# Autodesk Inventor assembly: 左後脚ユニット5
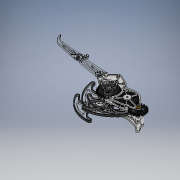
[picture p0: Inventor's stored thumbnail of the model, 180x180]
Saved by Autodesk Inventor 2020 (Build 240168000, 168)
## iProperties
Created: 2019-09-03
Part Number: 左後脚ユニット5
Document SubType Name: Assembly
Designer: 雪村
Mass: 251.015 g
Surface Area: 1556.42 cm^2
Volume: 120.818 cm^3
Density: 2.07763 g/cm^3
Author: 雪村
## Documents named in this file (29)
- C:\Users\white\Documents\SRDC\SRDC\Inventor_2017\2018年機体\2020年4年機体\左後脚ユニット5.iam
- C:\Users\white\Documents\SRDC\SRDC\Inventor_2017\2018年機体\2020年4年機体\脚クランク1.iam
- C:\Users\white\Documents\SRDC\SRDC\Inventor_2017\2018年機体\2020年4年機体\ヘッケン＋揺動節2.iam
- C:\Users\white\Documents\SRDC\SRDC\Inventor_2017\2018年機体\2020年4年機体\脚外フレーム5_MIR.ipt
- C:\Users\white\Documents\SRDC\SRDC\Inventor_2017\2018年機体\2020年4年機体\後脚ユニット締結パーツ5.ipt
- C:\Users\white\Documents\SRDC\SRDC\Inventor_2017\2018年機体\パーツ\スペーサーm3,40.ipt
- C:\Users\white\Documents\SRDC\SRDC\Inventor_2017\2018年機体\2020年4年機体\脚内フレーム5_MIR2.ipt
- C:\Users\white\Documents\SRDC\SRDC\Inventor_2017\2018年機体\2020年4年機体\脚最終段カム3.ipt
- C:\Users\white\Documents\SRDC\SRDC\Inventor_2017\2018年機体\パーツ\オイレスフランジ付き12142003.ipt
- C:\Users\white\Documents\SRDC\SRDC\Inventor_2017\2018年機体\パーツ\スペーサーm3,7.ipt
- C:\Users\white\Documents\SRDC\SRDC\Inventor_2017\2018年機体\2020年4年機体\歯車m2.z19.ipt
- C:\Users\white\Documents\SRDC\SRDC\Inventor_2017\2018年機体\パーツ\ベアリングフランジ付き0610.3t.ipt
- C:\Users\white\Documents\SRDC\SRDC\Inventor_2017\2018年機体\2020年4年機体\歯車m2.z25.ipt
- C:\Users\white\Documents\SRDC\SRDC\Inventor_2017\2018年機体\パーツ\オイレスフランジ付き06080512,1t ドライメット.ipt
- C:\Users\white\Documents\SRDC\SRDC\Inventor_2017\2018年機体\パーツ\スペーサーm3,6.ipt
- C:\Users\white\Documents\SRDC\SRDC\Inventor_2017\2018年機体\パーツ\ネジ鍋m3,12.ipt
- C:\Users\white\Documents\SRDC\SRDC\Inventor_2017\2018年機体\2020年4年機体\後脚ギアトレイン5.2.ipt
- C:\Users\white\Documents\SRDC\SRDC\Inventor_2017\2018年機体\2020年4年機体\歯車m2.z24.ipt
- C:\Users\white\Documents\SRDC\SRDC\Inventor_2017\2018年機体\2020年4年機体\後脚軸抑え1.ipt
- C:\Users\white\Documents\SRDC\SRDC\Inventor_2017\2018年機体\2020年4年機体\脚最終段カム4.ipt
- C:\Users\white\Documents\SRDC\SRDC\Inventor_2017\2018年機体\パーツ\スペーサーm3,4.ipt
- C:\Users\white\Documents\SRDC\SRDC\Inventor_2017\2018年機体\パーツ\ネジ皿m3,08.ipt
- C:\Users\white\Documents\SRDC\SRDC\Inventor_2017\2018年機体\パーツ\ネジ鍋m3,08.ipt
- C:\Users\white\Documents\SRDC\SRDC\Inventor_2017\2018年機体\パーツ\ネジ鍋m3,06.ipt
- C:\Users\white\Documents\SRDC\SRDC\Inventor_2017\2018年機体\パーツ\ネジ鍋m3,16.ipt
- C:\Users\white\Documents\SRDC\SRDC\Inventor_2017\2018年機体\2020年4年機体\後ウイング1.iam
- C:\Users\white\Documents\SRDC\SRDC\Inventor_2017\2018年機体\パーツ\スペーサーm3,20.ipt
- C:\Users\white\Documents\SRDC\SRDC\Inventor_2017\2018年機体\2020年4年機体\段ばね抑え2.ipt
- C:\Users\white\Documents\SRDC\SRDC\Inventor_2017\2018年機体\パーツ\スペーサーm3,5.ipt
## Components (75 placed, 28 different names)
1. 脚内フレーム5_MIR2:1 — 挿入:24, 挿入:25, 挿入:26, 挿入:27, 挿入:28, 挿入:39, 挿入:41, 挿入:43, 挿入:44, 挿入:45, 挿入:48, 挿入:62, 挿入:63, 挿入:64, 挿入:71, 挿入:72, 挿入:80, 挿入:85, 挿入:86, 挿入:87, 挿入:94
2. 脚クランク1:1 [sub-assembly] — 挿入:9, 挿入:10, 挿入:11, 挿入:12, 挿入:29, 挿入:30, 挿入:107
3. オイレスフランジ付き12142003:1 — 挿入:28
4. スペーサーm3,40:3 — 挿入:26
5. スペーサーm3,40:4 — 挿入:27, 挿入:70
6. スペーサーm3,40:2 — 挿入:25
7. スペーサーm3,40:1 — 挿入:24, 挿入:52, メイト:5
8. ヘッケン＋揺動節2:1 [sub-assembly] — 挿入:10
9. ヘッケン＋揺動節2:2 [sub-assembly] — 挿入:9
10. ヘッケン＋揺動節2:3 [sub-assembly] — 挿入:11
11. ヘッケン＋揺動節2:4 [sub-assembly] — 挿入:12
12. 脚外フレーム5_MIR:1 — 挿入:52, 挿入:70, 挿入:81, 挿入:82, 挿入:83, 挿入:84, 挿入:88, 挿入:106, 挿入:108
13. 後脚ユニット締結パーツ5:1 — メイト:5, 挿入:68, 挿入:69, 挿入:98, 挿入:99, 挿入:104, 挿入:105, 挿入:106
14. 脚最終段カム3:1 — 挿入:29, 挿入:30, 挿入:50, 挿入:51
15. スペーサーm3,7:1 — 挿入:48
16. スペーサーm3,7:2 — 挿入:39, 挿入:46
17. スペーサーm3,7:3 — 挿入:44
18. スペーサーm3,7:4 — 挿入:43
19. スペーサーm3,7:5 — 挿入:41, 挿入:47
20. 歯車m2.z19:1
21. ベアリングフランジ付き0610.3t:1
22. ベアリングフランジ付き0610.3t:2 — 挿入:72
23. 歯車m2.z25:1
24. ベアリングフランジ付き0610.3t:3 — 挿入:71
25. ベアリングフランジ付き0610.3t:4
26. オイレスフランジ付き06080512,1t ドライメット:1 — 挿入:45
27. オイレスフランジ付き06080512,1t ドライメット:2
28. スペーサーm3,6:1
29. スペーサーm3,6:2 — 挿入:49
30. ネジ鍋m3,12:1
31. ネジ鍋m3,12:2
32. 後脚ギアトレイン5.2:1 — 挿入:46, 挿入:47, 挿入:49, 挿入:73, 挿入:74, 挿入:75, 挿入:76
33. 歯車m2.z24:1 — 挿入:50, 挿入:51, 挿入:60, 挿入:61
34. 後脚軸抑え1:1 — 挿入:65, 挿入:66, 挿入:77, 挿入:78, 挿入:79
35. 脚最終段カム4:1 — 挿入:60, 挿入:61, 挿入:67, 挿入:89, 挿入:90, 挿入:91, 挿入:92
36. スペーサーm3,6:3 — 挿入:63, 挿入:66
37. スペーサーm3,6:4 — 挿入:62
38. スペーサーm3,6:5 — 挿入:64, 挿入:65
39. オイレスフランジ付き12142003:2 — 挿入:67
40. ベアリングフランジ付き0610.3t:5 — 挿入:68
41. スペーサーm3,4:1 — 挿入:69, 挿入:103
42. ネジ鍋m3,12:3 — 挿入:73
43. ネジ鍋m3,12:4 — 挿入:76
44. ネジ鍋m3,12:5 — 挿入:75
45. ネジ鍋m3,12:6 — 挿入:74
46. ネジ鍋m3,12:7 — 挿入:77
47. ネジ鍋m3,12:8 — 挿入:78
48. ネジ鍋m3,12:9 — 挿入:79
49. ネジ皿m3,08:1 — 挿入:80
50. ネジ鍋m3,08:1 — 挿入:86
51. ネジ鍋m3,08:2 — 挿入:87
52. ネジ鍋m3,08:3 — 挿入:85, 挿入:93
53. ネジ鍋m3,08:4 — 挿入:83
54. ネジ鍋m3,08:5 — 挿入:84
55. ネジ鍋m3,08:6 — 挿入:82
56. ネジ鍋m3,08:7 — 挿入:81
57. ネジ鍋m3,06:1 — 挿入:88
58. ネジ鍋m3,16:1 — 挿入:89
59. ネジ鍋m3,16:2 — 挿入:92
60. ネジ鍋m3,16:3 — 挿入:91
61. ネジ鍋m3,16:4 — 挿入:90
62. 後ウイング1:1 [sub-assembly] — 挿入:93
63. スペーサーm3,6:6 — 挿入:94
64. スペーサーm3,20:1 — 挿入:99
65. スペーサーm3,20:2
66. スペーサーm3,20:3 — 挿入:98
67. 段ばね抑え2:1 — 挿入:100, 挿入:101, 挿入:102
68. ネジ鍋m3,08:8 — 挿入:101
69. ネジ鍋m3,08:9 — 挿入:100
70. ネジ鍋m3,08:10 — 挿入:102
71. ネジ鍋m3,12:10 — 挿入:103
72. ネジ皿m3,08:2 — 挿入:104
73. ネジ皿m3,08:3 — 挿入:105
74. ベアリングフランジ付き0610.3t:6 — 挿入:108
75. スペーサーm3,5:1 — 挿入:107
## Relationships (86: Insert 81, Mate 5)
- [Insert]: 脚クランク1:1 ↔ オイレスフランジ付き12142003:1
- 挿入:9 [Insert] (0.5 mm): 脚クランク1:1 ↔ ヘッケン＋揺動節2:2
- 挿入:10 [Insert] (0.5 mm): 脚クランク1:1 ↔ ヘッケン＋揺動節2:1
- 挿入:11 [Insert] (0.5 mm): 脚クランク1:1 ↔ ヘッケン＋揺動節2:3
- 挿入:12 [Insert] (0.5 mm): 脚クランク1:1 ↔ ヘッケン＋揺動節2:4
- [Mate]: スペーサーm3,40:1 ↔ ヘッケン＋揺動節2:2
- [Mate]: スペーサーm3,40:1 ↔ ヘッケン＋揺動節2:1
- [Mate]: スペーサーm3,40:1 ↔ ヘッケン＋揺動節2:4
- [Mate]: スペーサーm3,40:1 ↔ ヘッケン＋揺動節2:3
- 挿入:24 [Insert]: 脚内フレーム5_MIR2:1 ↔ スペーサーm3,40:1
- 挿入:25 [Insert]: 脚内フレーム5_MIR2:1 ↔ スペーサーm3,40:2
- 挿入:26 [Insert]: 脚内フレーム5_MIR2:1 ↔ スペーサーm3,40:3
- 挿入:27 [Insert]: 脚内フレーム5_MIR2:1 ↔ スペーサーm3,40:4
- 挿入:28 [Insert]: 脚内フレーム5_MIR2:1 ↔ オイレスフランジ付き12142003:1
- 挿入:29 [Insert]: 脚クランク1:1 ↔ 脚最終段カム3:1
- 挿入:30 [Insert]: 脚クランク1:1 ↔ 脚最終段カム3:1
- [Insert]: 歯車m2.z19:1 ↔ ベアリングフランジ付き0610.3t:1
- [Insert]: 歯車m2.z19:1 ↔ ベアリングフランジ付き0610.3t:2
- [Insert]: 歯車m2.z25:1 ↔ ベアリングフランジ付き0610.3t:3
- [Insert]: 歯車m2.z25:1 ↔ ベアリングフランジ付き0610.3t:4
- [Insert]: オイレスフランジ付き06080512,1t ドライメット:1 ↔ ネジ鍋m3,12:1
- [Insert]: スペーサーm3,6:2 ↔ ネジ鍋m3,12:2
- [Insert]: オイレスフランジ付き06080512,1t ドライメット:2 ↔ スペーサーm3,6:2
- [Insert]: オイレスフランジ付き06080512,1t ドライメット:1 ↔ スペーサーm3,6:1
- 挿入:39 [Insert]: 脚内フレーム5_MIR2:1 ↔ スペーサーm3,7:2
- 挿入:41 [Insert]: 脚内フレーム5_MIR2:1 ↔ スペーサーm3,7:5
- 挿入:43 [Insert]: 脚内フレーム5_MIR2:1 ↔ スペーサーm3,7:4
- 挿入:44 [Insert]: 脚内フレーム5_MIR2:1 ↔ スペーサーm3,7:3
- 挿入:45 [Insert]: 脚内フレーム5_MIR2:1 ↔ オイレスフランジ付き06080512,1t ドライメット:1
- 挿入:46 [Insert]: スペーサーm3,7:2 ↔ 後脚ギアトレイン5.2:1
- 挿入:47 [Insert]: スペーサーm3,7:5 ↔ 後脚ギアトレイン5.2:1
- 挿入:48 [Insert]: 脚内フレーム5_MIR2:1 ↔ スペーサーm3,7:1
- 挿入:49 [Insert]: スペーサーm3,6:2 ↔ 後脚ギアトレイン5.2:1
- 挿入:50 [Insert]: 脚最終段カム3:1 ↔ 歯車m2.z24:1
- 挿入:51 [Insert]: 脚最終段カム3:1 ↔ 歯車m2.z24:1
- 挿入:52 [Insert]: スペーサーm3,40:1 ↔ 脚外フレーム5_MIR:1
- メイト:5 [Mate]: スペーサーm3,40:1 ↔ 後脚ユニット締結パーツ5:1
- 挿入:60 [Insert]: 歯車m2.z24:1 ↔ 脚最終段カム4:1
- 挿入:61 [Insert]: 歯車m2.z24:1 ↔ 脚最終段カム4:1
- 挿入:62 [Insert]: 脚内フレーム5_MIR2:1 ↔ スペーサーm3,6:4
- 挿入:63 [Insert]: 脚内フレーム5_MIR2:1 ↔ スペーサーm3,6:3
- 挿入:64 [Insert]: 脚内フレーム5_MIR2:1 ↔ スペーサーm3,6:5
- 挿入:65 [Insert]: 後脚軸抑え1:1 ↔ スペーサーm3,6:5
- 挿入:66 [Insert]: 後脚軸抑え1:1 ↔ スペーサーm3,6:3
- 挿入:67 [Insert]: 脚最終段カム4:1 ↔ オイレスフランジ付き12142003:2
- 挿入:68 [Insert]: 後脚ユニット締結パーツ5:1 ↔ ベアリングフランジ付き0610.3t:5
- 挿入:69 [Insert]: 後脚ユニット締結パーツ5:1 ↔ スペーサーm3,4:1
- 挿入:70 [Insert]: スペーサーm3,40:4 ↔ 脚外フレーム5_MIR:1
- 挿入:71 [Insert]: 脚内フレーム5_MIR2:1 ↔ ベアリングフランジ付き0610.3t:3
- 挿入:72 [Insert]: 脚内フレーム5_MIR2:1 ↔ ベアリングフランジ付き0610.3t:2
- 挿入:73 [Insert]: 後脚ギアトレイン5.2:1 ↔ ネジ鍋m3,12:3
- 挿入:74 [Insert]: 後脚ギアトレイン5.2:1 ↔ ネジ鍋m3,12:6
- 挿入:75 [Insert]: 後脚ギアトレイン5.2:1 ↔ ネジ鍋m3,12:5
- 挿入:76 [Insert]: 後脚ギアトレイン5.2:1 ↔ ネジ鍋m3,12:4
- 挿入:77 [Insert]: 後脚軸抑え1:1 ↔ ネジ鍋m3,12:7
- 挿入:78 [Insert]: 後脚軸抑え1:1 ↔ ネジ鍋m3,12:8
- 挿入:79 [Insert]: 後脚軸抑え1:1 ↔ ネジ鍋m3,12:9
- 挿入:80 [Insert]: 脚内フレーム5_MIR2:1 ↔ ネジ皿m3,08:1
- 挿入:81 [Insert]: 脚外フレーム5_MIR:1 ↔ ネジ鍋m3,08:7
- 挿入:82 [Insert]: 脚外フレーム5_MIR:1 ↔ ネジ鍋m3,08:6
- 挿入:83 [Insert]: 脚外フレーム5_MIR:1 ↔ ネジ鍋m3,08:4
- 挿入:84 [Insert]: 脚外フレーム5_MIR:1 ↔ ネジ鍋m3,08:5
- 挿入:85 [Insert]: 脚内フレーム5_MIR2:1 ↔ ネジ鍋m3,08:3
- 挿入:86 [Insert]: 脚内フレーム5_MIR2:1 ↔ ネジ鍋m3,08:1
- 挿入:87 [Insert]: 脚内フレーム5_MIR2:1 ↔ ネジ鍋m3,08:2
- 挿入:88 [Insert]: 脚外フレーム5_MIR:1 ↔ ネジ鍋m3,06:1
- 挿入:89 [Insert]: 脚最終段カム4:1 ↔ ネジ鍋m3,16:1
- 挿入:90 [Insert]: 脚最終段カム4:1 ↔ ネジ鍋m3,16:4
- 挿入:91 [Insert]: 脚最終段カム4:1 ↔ ネジ鍋m3,16:3
- 挿入:92 [Insert]: 脚最終段カム4:1 ↔ ネジ鍋m3,16:2
- 挿入:93 [Insert]: ネジ鍋m3,08:3 ↔ 後ウイング1:1
- 挿入:94 [Insert]: 脚内フレーム5_MIR2:1 ↔ スペーサーm3,6:6
- [Insert]: スペーサーm3,20:1 ↔ 段ばね抑え2:1
- [Insert]: スペーサーm3,20:2 ↔ 段ばね抑え2:1
- [Insert]: スペーサーm3,20:3 ↔ 段ばね抑え2:1
- 挿入:98 [Insert]: 後脚ユニット締結パーツ5:1 ↔ スペーサーm3,20:3
- 挿入:99 [Insert]: 後脚ユニット締結パーツ5:1 ↔ スペーサーm3,20:1
- 挿入:100 [Insert]: 段ばね抑え2:1 ↔ ネジ鍋m3,08:9
- 挿入:101 [Insert]: 段ばね抑え2:1 ↔ ネジ鍋m3,08:8
- 挿入:102 [Insert]: 段ばね抑え2:1 ↔ ネジ鍋m3,08:10
- 挿入:103 [Insert]: スペーサーm3,4:1 ↔ ネジ鍋m3,12:10
- 挿入:104 [Insert]: 後脚ユニット締結パーツ5:1 ↔ ネジ皿m3,08:2
- 挿入:105 [Insert]: 後脚ユニット締結パーツ5:1 ↔ ネジ皿m3,08:3
- 挿入:106 [Insert]: 脚外フレーム5_MIR:1 ↔ 後脚ユニット締結パーツ5:1
- 挿入:107 [Insert]: 脚クランク1:1 ↔ スペーサーm3,5:1
- 挿入:108 [Insert]: 脚外フレーム5_MIR:1 ↔ ベアリングフランジ付き0610.3t:6
## Named parameters: d0_d2 = 0 mm, d6_d1 = 0 mm, d7_d0 = 0 mm, d43_d9 = 0 mm, d44_d10 = 0 mm, d108_d98 = 0 mm, d109_d99 = 0 mm, d110_d100 = 0 mm
